# Autodesk Inventor assembly: Arm 1.1
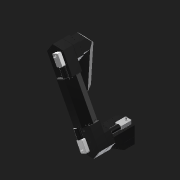
[picture p0: Inventor's stored thumbnail of the model, 180x180]
Saved by Autodesk Inventor 2017 (Build 210142000, 142)
## iProperties
Created: 2019-09-19
Part Number: Arm 1.1
Document SubType Name: Assembly
Designer: Dell
Author: Dell
## Documents named in this file (4)
- C:\Users\Dell\Documents\GitHub\tr2\Arm 1.1\Arm 1.1.iam
- C:\Users\Dell\Documents\GitHub\tr2\Actuator 1.6\Actuator 1.6.iam
- C:\Users\Dell\Documents\GitHub\tr2\Arm 1.1\A01.ipt
- C:\Users\Dell\Documents\GitHub\tr2\Arm 1.1\A02.ipt
## Components (5 placed, 3 different names)
1. Actuator 1.6:1 [sub-assembly] — Mate:1, Mate:2
2. Actuator 1.6:2 [sub-assembly] — Mate:1, Mate:2, Mate:5, Mate:8, Mate:9, Mate:10
3. A01:1 — Mate:5, Mate:8, Mate:9, Mate:10, Mate:11, Mate:12, Mate:13, Mate:14
4. Actuator 1.6:3 [sub-assembly] — Mate:11, Mate:12, Mate:13, Mate:14, Mate:15, Mate:16
5. A02:1 — Mate:15, Mate:16
## Relationships (12: Mate 12)
- Mate:1: Actuator 1.6:1 ↔ Actuator 1.6:2
- Mate:2: Actuator 1.6:1 ↔ Actuator 1.6:2
- Mate:5: Actuator 1.6:2 ↔ A01:1
- Mate:8: Actuator 1.6:2 ↔ A01:1
- Mate:9: Actuator 1.6:2 ↔ A01:1
- Mate:10: Actuator 1.6:2 ↔ A01:1
- Mate:11: A01:1 ↔ Actuator 1.6:3
- Mate:12: A01:1 ↔ Actuator 1.6:3
- Mate:13: A01:1 ↔ Actuator 1.6:3
- Mate:14: A01:1 ↔ Actuator 1.6:3
- Mate:15: Actuator 1.6:3 ↔ A02:1
- Mate:16: Actuator 1.6:3 ↔ A02:1
